# Autodesk Inventor assembly: JukeBox SQ
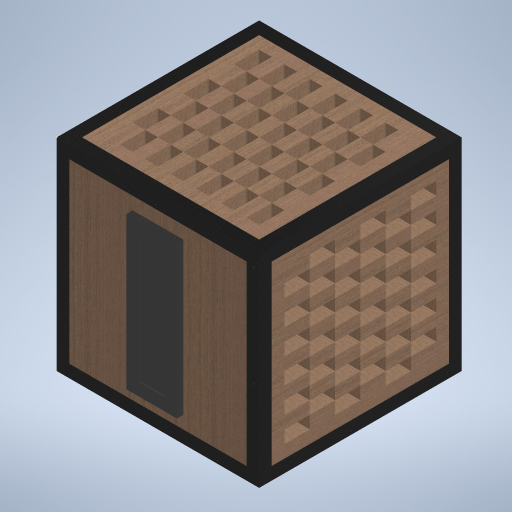
[picture p0: Inventor's stored thumbnail of the model, 512x512]
Saved by Autodesk Inventor 2024 (Build 280153000, 153)
## iProperties
Created: 2023-04-26
Part Number: JukeBox SQ
Document SubType Name: Assembly
Designer: newic
Author: newic
## Documents named in this file (6)
- D:\.My Models\.Inventor\Jukebox Project\JukeBox SQ.iam
- D:\.My Models\.Inventor\Jukebox Project\JukeBox Metal Frame.ipt
- D:\.My Models\.Inventor\Jukebox Project\JukeBox Outside panel sharp edges.ipt
- D:\.My Models\.Inventor\Jukebox Project\JukeBox Bottem Panel.ipt
- D:\.My Models\.Inventor\Jukebox Project\JukeBox CD Player SQ.ipt
- D:\.My Models\.Inventor\Jukebox Project\JukeBox Top Panel SQ.ipt
## Components (8 placed, 5 different names)
1. JukeBox Metal Frame:1 — Mate:3, Mate:4, Mate:5, Mate:6, Mate:7, Mate:8, Mate:9, Mate:10, Mate:11, Mate:12, Flush:1, Flush:2, Flush:3, Flush:4, Flush:5, Mate:13, Mate:14, Flush:6
2. JukeBox Outside panel sharp edges:1 — Mate:3, Mate:4, Flush:2
3. JukeBox Outside panel sharp edges:2 — Mate:7, Mate:8, Flush:4
4. JukeBox Outside panel sharp edges:3 — Mate:5, Mate:6, Flush:3
5. JukeBox Outside panel sharp edges:4 — Mate:9, Mate:10, Flush:1
6. JukeBox Bottem Panel:1 — Mate:11, Mate:12, Flush:5, Mate:17
7. JukeBox CD Player SQ:1 — Mate:15, Mate:16, Mate:17
8. JukeBox Top Panel SQ:1 — Mate:13, Mate:14, Flush:6, Mate:15, Mate:16
## Relationships (21: Mate 15, Flush 6)
- Mate:3: JukeBox Metal Frame:1 ↔ JukeBox Outside panel sharp edges:1
- Mate:4: JukeBox Metal Frame:1 ↔ JukeBox Outside panel sharp edges:1
- Mate:5: JukeBox Metal Frame:1 ↔ JukeBox Outside panel sharp edges:3
- Mate:6: JukeBox Metal Frame:1 ↔ JukeBox Outside panel sharp edges:3
- Mate:7: JukeBox Metal Frame:1 ↔ JukeBox Outside panel sharp edges:2
- Mate:8: JukeBox Metal Frame:1 ↔ JukeBox Outside panel sharp edges:2
- Mate:9: JukeBox Metal Frame:1 ↔ JukeBox Outside panel sharp edges:4
- Mate:10: JukeBox Metal Frame:1 ↔ JukeBox Outside panel sharp edges:4
- Mate:11: JukeBox Metal Frame:1 ↔ JukeBox Bottem Panel:1
- Mate:12: JukeBox Metal Frame:1 ↔ JukeBox Bottem Panel:1
- Flush:1: JukeBox Metal Frame:1 ↔ JukeBox Outside panel sharp edges:4
- Flush:2: JukeBox Metal Frame:1 ↔ JukeBox Outside panel sharp edges:1
- Flush:3: JukeBox Metal Frame:1 ↔ JukeBox Outside panel sharp edges:3
- Flush:4: JukeBox Metal Frame:1 ↔ JukeBox Outside panel sharp edges:2
- Flush:5: JukeBox Metal Frame:1 ↔ JukeBox Bottem Panel:1
- Mate:13: JukeBox Metal Frame:1 ↔ JukeBox Top Panel SQ:1
- Mate:14: JukeBox Metal Frame:1 ↔ JukeBox Top Panel SQ:1
- Flush:6: JukeBox Metal Frame:1 ↔ JukeBox Top Panel SQ:1
- Mate:15: JukeBox CD Player SQ:1 ↔ JukeBox Top Panel SQ:1
- Mate:16: JukeBox CD Player SQ:1 ↔ JukeBox Top Panel SQ:1
- Mate:17: JukeBox Bottem Panel:1 ↔ JukeBox CD Player SQ:1
